# Autodesk Inventor assembly: Base1
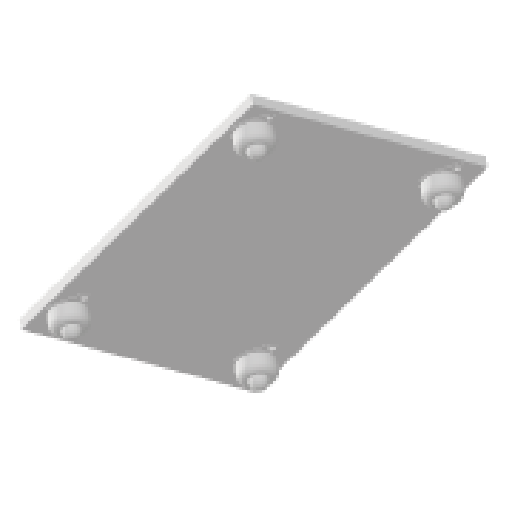
[picture p0: Inventor's stored thumbnail of the model, 512x512]
Saved by Autodesk Inventor 2024 (Build 280153000, 153)
## iProperties
Created: 2024-03-16
Part Number: Base1
Document SubType Name: Assembly
Designer: op04o
Author: op04o
## Documents named in this file (3)
- C:\Users\op04o\OneDrive\桌面\實務\Base\Base1.iam
- C:\Users\op04o\OneDrive\桌面\實務\Base\base.ipt
- C:\Users\op04o\OneDrive\桌面\實務\Base\cow_wheel.ipt
## Components (5 placed, 2 different names)
1. base:1 — Insert:1, Insert:2, Insert:3, Insert:4, Insert:5, Insert:6, Insert:7, Insert:8
2. cow_wheel:1 — Insert:3, Insert:4
3. cow_wheel:2 — Insert:7, Insert:8
4. cow_wheel:3 — Insert:1, Insert:2
5. cow_wheel:4 — Insert:5, Insert:6
## Relationships (8: Insert 8)
- Insert:1: base:1 ↔ cow_wheel:3
- Insert:2: base:1 ↔ cow_wheel:3
- Insert:3: base:1 ↔ cow_wheel:1
- Insert:4: base:1 ↔ cow_wheel:1
- Insert:5: base:1 ↔ cow_wheel:4
- Insert:6: base:1 ↔ cow_wheel:4
- Insert:7: base:1 ↔ cow_wheel:2
- Insert:8: base:1 ↔ cow_wheel:2
